# Autodesk Inventor assembly: Shoulder
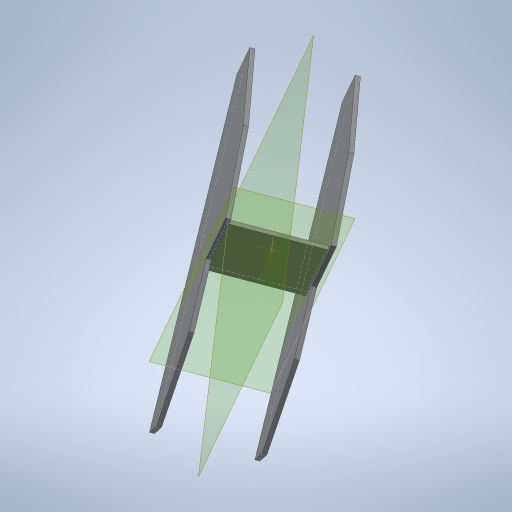
[picture p0: Inventor's stored thumbnail of the model, 512x512]
Saved by Autodesk Inventor 2023 (Build 270158000, 158)
## iProperties
Created: 2020-03-24
Part Number: Shoulder
Document SubType Name: Assembly
Designer: valer
Mass: 4853.13 g
Surface Area: 3141.52 cm^2
Volume: 1403.99 cm^3
Density: 3.45667 g/cm^3
Author: valer
## Documents named in this file (6)
- C:\Users\LattePanda\Desktop\str1ker\description\models\src\Shoulder.iam
- C:\Users\LattePanda\Desktop\str1ker\parts\UpperArmBracket.ipt
- C:\Users\LattePanda\Desktop\str1ker\parts\external\ShoulderMiterGear.ipt
- C:\Users\LattePanda\Desktop\str1ker\parts\external\ServoShaft.ipt
- C:\Users\LattePanda\Desktop\str1ker\parts\external\Shoulder6mmDShaftHub-545578.ipt
- C:\Users\LattePanda\Desktop\str1ker\description\models\src\ShoulderBoundingBox.ipt
## Components (7 placed, 5 different names)
1. UpperArmBracket:5
2. UpperArmBracket:6 — Angle:1
3. ShoulderMiterGear:2 — Mate:382
4. ShoulderServoShaft:2 — Mate:374, Mate:382, Flush:1
5. Shoulder6mmDShaftHub-545578:1 — Mate:374, Flush:1
6. Shoulder6mmDShaftHub-545578:2
7. ShoulderBoundingBox:1 — Mate:386, Flush:6, Flush:7
## Relationships (7: Mate 3, Flush 3, Angle 1)
- Mate:374: ShoulderServoShaft:2 ↔ Shoulder6mmDShaftHub-545578:1
- Mate:382: ShoulderMiterGear:2 ↔ ShoulderServoShaft:2
- Flush:1 (-4 mm): ShoulderServoShaft:2 ↔ Shoulder6mmDShaftHub-545578:1
- Angle:1 (0 deg): UpperArmBracket:6
- Mate:386: ShoulderBoundingBox:1
- Flush:6: ShoulderBoundingBox:1
- Flush:7: ShoulderBoundingBox:1
